# Autodesk Inventor assembly: AMR_Full_System_V1
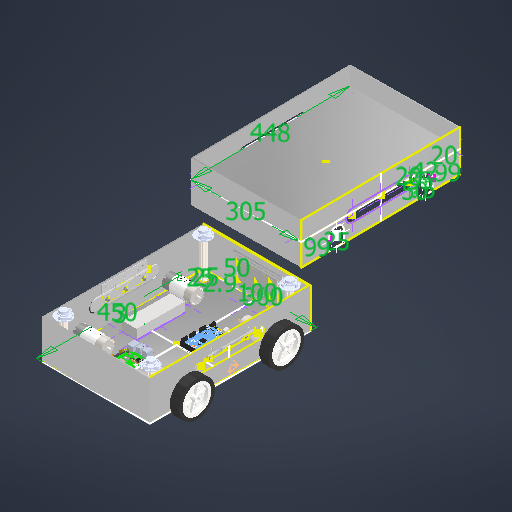
[picture p0: Inventor's stored thumbnail of the model, 512x512]
Saved by Autodesk Inventor 2026.2 (Build 302298010, 298A)
## iProperties
Created: 2026-03-25
Part Number: AMR_Full_System_V1
Document SubType Name: Assembly
Designer: Srishanth Dhondy
Author: Srishanth Dhondy
## Documents named in this file (27)
- D:\Cloud_Downloads\Srishanth\My Folder\Projects\AMR\CAD Design\hardware_cad\AMR_Full_System_V1.iam
- D:\Cloud_Downloads\Srishanth\My Folder\Projects\AMR\CAD Design\hardware_cad\AMR_Base_Box_V2.ipt
- D:\Cloud_Downloads\Srishanth\My Folder\Projects\AMR\CAD Design\hardware_cad\AMR_Top_Basket.ipt
- D:\Cloud_Downloads\Srishanth\My Folder\Projects\AMR\CAD Design\hardware_cad\Grab CAD\Wheels\Wheels v8\Wheels v8\Wheels v8.ipt
- D:\Cloud_Downloads\Srishanth\My Folder\Projects\AMR\CAD Design\hardware_cad\Grab CAD\orange-planetary-gear-dc-motor-12v-970-rpm-14-5-n-cm-pg36m555-5-2k-1.snapshot.2\Motor\Motor\Motor.ipt
- D:\Cloud_Downloads\Srishanth\My Folder\Projects\AMR\CAD Design\hardware_cad\Grab CAD\T-Slot\Aluminum Extrusion Bar\Aluminum Extrusion Bar\Aluminum Extrusion Bar.ipt
- D:\Cloud_Downloads\Srishanth\My Folder\Projects\AMR\CAD Design\hardware_cad\Grab CAD\Raspberry Pi 4\Raspberry Pi 4 Model B\Raspberry Pi 4 Model B\Raspberry Pi 4 Model B.ipt
- D:\Cloud_Downloads\Srishanth\My Folder\Projects\AMR\CAD Design\hardware_cad\AMR_Handle_Flap.ipt
- D:\Cloud_Downloads\Srishanth\My Folder\Projects\AMR\CAD Design\hardware_cad\LiPo_Battery_Dummy.ipt
- D:\Cloud_Downloads\Srishanth\My Folder\Projects\AMR\CAD Design\hardware_cad\Rear_Port_Slider.ipt
- D:\Cloud_Downloads\Srishanth\My Folder\Projects\AMR\CAD Design\hardware_cad\Grab CAD\50kg_Load_Sensor\assembly\assembly\assembly.iam
- D:\Cloud_Downloads\Srishanth\My Folder\Projects\AMR\CAD Design\hardware_cad\15205A113_Spring Hinge\15205A113_Spring Hinge\Dynamic_Hinge.iam
- C:\Users\Srishanth Dhondy\Documents\Inventor\Content Center Files\R2026\en-US\ISO 7089\ISO 7089 - 2.5 - 140 HV(1).ipt
- C:\Users\Srishanth Dhondy\Documents\Inventor\Content Center Files\R2026\en-US\ISO 4762(2)\ISO 4762 - M2.5 x 10ISO.ipt
- C:\Users\Srishanth Dhondy\Documents\Inventor\Content Center Files\R2026\en-US\ISO 7089\ISO 7089 - 3.5 - 140 HV(1).ipt
- C:\Users\Srishanth Dhondy\Documents\Inventor\Content Center Files\R2026\en-US\ISO 4762(2)\ISO 4762 - M3 x 10ISO.ipt
- C:\Users\Srishanth Dhondy\Documents\Inventor\Content Center Files\R2026\en-US\ISO 7089\ISO 7089 - 4 - 140 HV(1).ipt
- C:\Users\Srishanth Dhondy\Documents\Inventor\Content Center Files\R2026\en-US\ISO 4762(2)\ISO 4762 - M4 x 12ISO.ipt
- C:\Users\Srishanth Dhondy\Documents\Inventor\Content Center Files\R2026\en-US\DIN 985\DIN 985 - M4.ipt
- D:\Cloud_Downloads\Srishanth\My Folder\Projects\AMR\CAD Design\hardware_cad\Grab CAD\Arduino\Arduino Mega 2560 R3 v23\Arduino Mega 2560 R3 v23\Arduino Mega 2560 R3 v23.ipt
- C:\Users\Srishanth Dhondy\Documents\Inventor\Content Center Files\R2026\en-US\ISO 4762(2)\ISO 4762 - M2.5 x 16ISO.ipt
- C:\Users\Srishanth Dhondy\Documents\Inventor\Content Center Files\R2026\en-US\ISO 4032(2)\ISO 4032 - M2.5 - ISO.ipt
- D:\Cloud_Downloads\Srishanth\My Folder\Projects\AMR\CAD Design\hardware_cad\AMR_Full_System_V1\AIP\FEA\fg5kdr8u8.fins
- D:\Cloud_Downloads\Srishanth\My Folder\Projects\AMR\CAD Design\hardware_cad\AMR_Full_System_V1\AIP\FEA\fg5kdr8u8.fsat
- D:\Cloud_Downloads\Srishanth\My Folder\Projects\AMR\CAD Design\hardware_cad\AMR_Full_System_V1\AIP\FEA\fg5kdr8u8.ftes
- D:\Cloud_Downloads\Srishanth\My Folder\Projects\AMR\CAD Design\hardware_cad\AMR_Full_System_V1\AIP\FEA\fg5kdr8u8.fwiz
- D:\Cloud_Downloads\Srishanth\My Folder\Projects\AMR\CAD Design\hardware_cad\AMR_Full_System_V1\AIP\FEA\fg5kdseqo.fmsh
## Components (107 placed, 21 different names)
1. AMR_Base_Box_V2:1 — Mate:1, Rigid:11, Rigid:12, Rigid:13, Rigid:14, Slider:17, Rigid:15, Rotational:7, Rotational:8, Insert:1, Insert:2, Insert:3, Insert:4, Mate:2, Mate:4, Mate:6, Mate:8, Rotational:11, Insert:5, Insert:6, Insert:7, Insert:8, Insert:9, Insert:10, Insert:11, Insert:12, Rotational:13, Rotational:15, Insert:21, Insert:22, Insert:23, Insert:24, Insert:25, Insert:26, Insert:27, Insert:28, Rotational:19, Rotational:21, Rotational:22, Insert:63, Insert:64, Insert:65, Insert:66
2. AMR_Top_Basket:1
3. Aluminum Extrusion Bar:2 — Rigid:13, Rotational:24
4. Aluminum Extrusion Bar:3 — Rigid:12, Rigid:20
5. Aluminum Extrusion Bar:5 — Rigid:11, Rotational:25
6. Wheels v8:6
7. Raspberry Pi 4 Model B:1 — Rotational:23, Insert:71, Insert:72, Insert:73, Insert:74
8. AMR_Handle_Flap:1 — Rigid:17, Insert:43, Insert:44, Insert:45, Rigid:19
9. AMR_Handle_Flap:2 — Rotational:6, Rigid:16, Rigid:18, Insert:57, Insert:58, Insert:59
10. LiPo_Battery_Dummy:1 — Rotational:22
11. Aluminum Extrusion Bar:6 — Rigid:14, Rigid:21
12. Dynamic_Hinge:1 [sub-assembly] — Rigid:15, Rotational:6, Rigid:16, Rigid:18, Insert:51, Insert:52, Insert:53
13. Rear_Port_Slider:2 — Slider:17
14. Dynamic_Hinge:2 [sub-assembly] — Rotational:7, Rotational:8, Rigid:17, Insert:37, Insert:38, Insert:39, Rigid:19
15. ISO 7089 2.5:1 — Insert:1, Mate:3, Mate:5, Mate:7, Mate:9
16. ISO 7089 2.5:2 — Insert:2
17. ISO 7089 2.5:3 — Insert:3
18. ISO 7089 2.5:4 — Insert:4
19. ISO 4762 M2.5 x 10:1 — Mate:2, Mate:3
20. ISO 4762 M2.5 x 10:2 — Mate:4, Mate:5
21. ISO 4762 M2.5 x 10:3 — Mate:6, Mate:7
22. ISO 4762 M2.5 x 10:4 — Mate:8, Mate:9
23. Motor:5 — Rotational:11, Rotational:12
24. ISO 7089 3.5:1 — Insert:5, Insert:16
25. ISO 7089 3.5:2 — Insert:6, Insert:14
26. ISO 7089 3.5:3 — Insert:7, Insert:17
27. ISO 7089 3.5:4 — Insert:8, Insert:18
28. ISO 7089 3.5:5 — Insert:9, Insert:13
29. ISO 7089 3.5:6 — Insert:10, Insert:15
30. ISO 7089 3.5:7 — Insert:11, Insert:20
31. ISO 7089 3.5:8 — Insert:12, Insert:19
32. ISO 4762 M3 x 10:1 — Insert:13
33. ISO 4762 M3 x 10:2 — Insert:14
34. ISO 4762 M3 x 10:3 — Insert:15
35. ISO 4762 M3 x 10:4 — Insert:16
36. Wheels v8:7 — Rotational:12
37. Motor:7 — Rotational:13, Rotational:14
38. Motor:8 — Rotational:15, Rotational:16
39. ISO 4762 M3 x 10:5 — Insert:17
40. ISO 4762 M3 x 10:6 — Insert:18
41. ISO 4762 M3 x 10:7 — Insert:19
42. ISO 4762 M3 x 10:8 — Insert:20
43. Wheels v8:8 — Rotational:14
44. ISO 7089 3.5:9 — Insert:21, Insert:29
45. ISO 7089 3.5:10 — Insert:22, Insert:32
46. ISO 7089 3.5:11 — Insert:23, Insert:34
47. ISO 7089 3.5:12 — Insert:24, Insert:33
48. ISO 7089 3.5:13 — Insert:25, Insert:31
49. ISO 7089 3.5:14 — Insert:26, Insert:30
50. ISO 7089 3.5:15 — Insert:27, Insert:36
51. ISO 7089 3.5:16 — Insert:28, Insert:35
52. ISO 4762 M3 x 10:9 — Insert:29
53. ISO 4762 M3 x 10:10 — Insert:30
54. ISO 4762 M3 x 10:11 — Insert:31
55. ISO 4762 M3 x 10:12 — Insert:32
56. Wheels v8:10 — Rotational:20
57. Motor:9 — Rotational:19, Rotational:20
58. Wheels v8:11 — Rotational:16
59. ISO 4762 M3 x 10:13 — Insert:33
60. ISO 4762 M3 x 10:14 — Insert:34
61. ISO 4762 M3 x 10:15 — Insert:35
62. ISO 4762 M3 x 10:16 — Insert:36
63. ISO 7089 4:1 — Insert:37, Insert:40
64. ISO 7089 4:2 — Insert:38, Insert:42
65. ISO 7089 4:3 — Insert:39, Insert:41
66. ISO 4762 M4 x 12:1 — Insert:40
67. ISO 4762 M4 x 12:2 — Insert:41
68. ISO 4762 M4 x 12:3 — Insert:42
69. ISO 7089 4:4 — Insert:43, Insert:49
70. ISO 7089 4:5 — Insert:44, Insert:50
71. ISO 7089 4:6 — Insert:45, Insert:48
72. DIN 985 - replaced by DIN EN ISO 10511 M4:3 — Insert:48
73. DIN 985 - replaced by DIN EN ISO 10511 M4:5 — Insert:49
74. DIN 985 - replaced by DIN EN ISO 10511 M4:6 — Insert:50
75. ISO 7089 4:7 — Insert:51, Insert:54
76. ISO 7089 4:8 — Insert:52, Insert:55
77. ISO 7089 4:9 — Insert:53, Insert:56
78. ISO 4762 M4 x 12:4 — Insert:54
79. ISO 4762 M4 x 12:5 — Insert:55
80. ISO 4762 M4 x 12:6 — Insert:56
81. ISO 7089 4:10 — Insert:57, Insert:60
82. ISO 7089 4:11 — Insert:58, Insert:61
83. ISO 7089 4:12 — Insert:59, Insert:62
84. DIN 985 - replaced by DIN EN ISO 10511 M4:7 — Insert:60
85. DIN 985 - replaced by DIN EN ISO 10511 M4:8 — Insert:61
86. DIN 985 - replaced by DIN EN ISO 10511 M4:9 — Insert:62
87. Arduino Mega 2560 R3 v23:1 — Rotational:21
88. ISO 7089 2.5:5 — Insert:63, Insert:67
89. ISO 7089 2.5:6 — Insert:64, Insert:70
90. ISO 7089 2.5:7 — Insert:65, Insert:68
91. ISO 7089 2.5:8 — Insert:66, Insert:69
92. ISO 4762 M2.5 x 16:1 — Insert:67
93. ISO 4762 M2.5 x 16:2 — Insert:68, Rotational:23
94. ISO 4762 M2.5 x 16:3 — Insert:69
95. ISO 4762 M2.5 x 16:4 — Insert:70
96. ISO 7089 2.5:9 — Insert:71, Insert:75
97. ISO 7089 2.5:10 — Insert:72, Insert:76
98. ISO 7089 2.5:11 — Insert:73, Insert:77
99. ISO 7089 2.5:12 — Insert:74, Insert:78
100. ISO 4032 M2.5:1 — Insert:75
101. ISO 4032 M2.5:2 — Insert:76
102. ISO 4032 M2.5:3 — Insert:77
103. ISO 4032 M2.5:4 — Insert:78
104. assembly:5 [sub-assembly] — Rotational:24
105. assembly:6 [sub-assembly] — Rotational:25
106. assembly:7 [sub-assembly] — Rigid:21
107. assembly:8 [sub-assembly] — Rigid:20
## Relationships (114: Insert 76, RevoluteJoint 16, WeldJoint 11, Mate 9, Flush 1, TranslationJoint 1)
- Mate:1: AMR_Base_Box_V2:1
- Flush:1 (-55 mm)
- Rigid:11 [WeldJoint]: AMR_Base_Box_V2:1 ↔ Aluminum Extrusion Bar:5
- Rigid:12 [WeldJoint]: AMR_Base_Box_V2:1 ↔ Aluminum Extrusion Bar:3
- Rigid:13 [WeldJoint]: AMR_Base_Box_V2:1 ↔ Aluminum Extrusion Bar:2
- Rigid:14 [WeldJoint]: AMR_Base_Box_V2:1 ↔ Aluminum Extrusion Bar:6
- Slider:17 [TranslationJoint]: AMR_Base_Box_V2:1 ↔ Rear_Port_Slider:2
- Rigid:15 [WeldJoint]: AMR_Base_Box_V2:1 ↔ Dynamic_Hinge:1
- Rotational:6 [RevoluteJoint]: AMR_Handle_Flap:2 ↔ Dynamic_Hinge:1
- Rigid:16 [WeldJoint]: AMR_Handle_Flap:2 ↔ Dynamic_Hinge:1
- Rotational:7 [RevoluteJoint]: AMR_Base_Box_V2:1 ↔ Dynamic_Hinge:2
- Rotational:8 [RevoluteJoint]: AMR_Base_Box_V2:1 ↔ Dynamic_Hinge:2
- Rigid:17 [WeldJoint]: AMR_Handle_Flap:1 ↔ Dynamic_Hinge:2
- Insert:1: AMR_Base_Box_V2:1 ↔ ISO 7089 2.5:1
- Insert:2: AMR_Base_Box_V2:1 ↔ ISO 7089 2.5:2
- Insert:3: AMR_Base_Box_V2:1 ↔ ISO 7089 2.5:3
- Insert:4: AMR_Base_Box_V2:1 ↔ ISO 7089 2.5:4
- Mate:2: AMR_Base_Box_V2:1 ↔ ISO 4762 M2.5 x 10:1
- Mate:3: ISO 7089 2.5:1 ↔ ISO 4762 M2.5 x 10:1
- Mate:4: AMR_Base_Box_V2:1 ↔ ISO 4762 M2.5 x 10:2
- Mate:5: ISO 7089 2.5:1 ↔ ISO 4762 M2.5 x 10:2
- Mate:6: AMR_Base_Box_V2:1 ↔ ISO 4762 M2.5 x 10:3
- Mate:7: ISO 7089 2.5:1 ↔ ISO 4762 M2.5 x 10:3
- Mate:8: AMR_Base_Box_V2:1 ↔ ISO 4762 M2.5 x 10:4
- Mate:9: ISO 7089 2.5:1 ↔ ISO 4762 M2.5 x 10:4
- Rotational:11 [RevoluteJoint]: AMR_Base_Box_V2:1 ↔ Motor:5
- Insert:5: AMR_Base_Box_V2:1 ↔ ISO 7089 3.5:1
- Insert:6: AMR_Base_Box_V2:1 ↔ ISO 7089 3.5:2
- Insert:7: AMR_Base_Box_V2:1 ↔ ISO 7089 3.5:3
- Insert:8: AMR_Base_Box_V2:1 ↔ ISO 7089 3.5:4
- Insert:9: AMR_Base_Box_V2:1 ↔ ISO 7089 3.5:5
- Insert:10: AMR_Base_Box_V2:1 ↔ ISO 7089 3.5:6
- Insert:11: AMR_Base_Box_V2:1 ↔ ISO 7089 3.5:7
- Insert:12: AMR_Base_Box_V2:1 ↔ ISO 7089 3.5:8
- Insert:13: ISO 7089 3.5:5 ↔ ISO 4762 M3 x 10:1
- Insert:14: ISO 7089 3.5:2 ↔ ISO 4762 M3 x 10:2
- Insert:15: ISO 7089 3.5:6 ↔ ISO 4762 M3 x 10:3
- Insert:16: ISO 7089 3.5:1 ↔ ISO 4762 M3 x 10:4
- Rotational:12 [RevoluteJoint]: Motor:5 ↔ Wheels v8:7
- Rotational:13 [RevoluteJoint]: AMR_Base_Box_V2:1 ↔ Motor:7
- Insert:17: ISO 7089 3.5:3 ↔ ISO 4762 M3 x 10:5
- Insert:18: ISO 7089 3.5:4 ↔ ISO 4762 M3 x 10:6
- Insert:19: ISO 7089 3.5:8 ↔ ISO 4762 M3 x 10:7
- Insert:20: ISO 7089 3.5:7 ↔ ISO 4762 M3 x 10:8
- Rotational:14 [RevoluteJoint]: Motor:7 ↔ Wheels v8:8
- Rotational:15 [RevoluteJoint]: AMR_Base_Box_V2:1 ↔ Motor:8
- Insert:21: AMR_Base_Box_V2:1 ↔ ISO 7089 3.5:9
- Insert:22: AMR_Base_Box_V2:1 ↔ ISO 7089 3.5:10
- Insert:23: AMR_Base_Box_V2:1 ↔ ISO 7089 3.5:11
- Insert:24: AMR_Base_Box_V2:1 ↔ ISO 7089 3.5:12
- Insert:25: AMR_Base_Box_V2:1 ↔ ISO 7089 3.5:13
- Insert:26: AMR_Base_Box_V2:1 ↔ ISO 7089 3.5:14
- Insert:27: AMR_Base_Box_V2:1 ↔ ISO 7089 3.5:15
- Insert:28: AMR_Base_Box_V2:1 ↔ ISO 7089 3.5:16
- Insert:29: ISO 7089 3.5:9 ↔ ISO 4762 M3 x 10:9
- Insert:30: ISO 7089 3.5:14 ↔ ISO 4762 M3 x 10:10
- Insert:31: ISO 7089 3.5:13 ↔ ISO 4762 M3 x 10:11
- Insert:32: ISO 7089 3.5:10 ↔ ISO 4762 M3 x 10:12
- Rotational:16 [RevoluteJoint]: Motor:8 ↔ Wheels v8:11
- Rotational:19 [RevoluteJoint]: AMR_Base_Box_V2:1 ↔ Motor:9
- Insert:33: ISO 7089 3.5:12 ↔ ISO 4762 M3 x 10:13
- Insert:34: ISO 7089 3.5:11 ↔ ISO 4762 M3 x 10:14
- Insert:35: ISO 7089 3.5:16 ↔ ISO 4762 M3 x 10:15
- Insert:36: ISO 7089 3.5:15 ↔ ISO 4762 M3 x 10:16
- Rotational:20 [RevoluteJoint]: Wheels v8:10 ↔ Motor:9
- Insert:37: Dynamic_Hinge:2 ↔ ISO 7089 4:1
- Insert:38: Dynamic_Hinge:2 ↔ ISO 7089 4:2
- Insert:39: Dynamic_Hinge:2 ↔ ISO 7089 4:3
- Insert:40: ISO 7089 4:1 ↔ ISO 4762 M4 x 12:1
- Insert:41: ISO 7089 4:3 ↔ ISO 4762 M4 x 12:2
- Insert:42: ISO 7089 4:2 ↔ ISO 4762 M4 x 12:3
- Insert:43: AMR_Handle_Flap:1 ↔ ISO 7089 4:4
- Insert:44: AMR_Handle_Flap:1 ↔ ISO 7089 4:5
- Insert:45: AMR_Handle_Flap:1 ↔ ISO 7089 4:6
- Insert:48: ISO 7089 4:6 ↔ DIN 985 - replaced by DIN EN ISO 10511 M4:3
- Insert:49: ISO 7089 4:4 ↔ DIN 985 - replaced by DIN EN ISO 10511 M4:5
- Insert:50: ISO 7089 4:5 ↔ DIN 985 - replaced by DIN EN ISO 10511 M4:6
- Rigid:18 [WeldJoint]: AMR_Handle_Flap:2 ↔ Dynamic_Hinge:1
- Rigid:19 [WeldJoint]: AMR_Handle_Flap:1 ↔ Dynamic_Hinge:2
- Insert:51: Dynamic_Hinge:1 ↔ ISO 7089 4:7
- Insert:52: Dynamic_Hinge:1 ↔ ISO 7089 4:8
- Insert:53: Dynamic_Hinge:1 ↔ ISO 7089 4:9
- Insert:54: ISO 7089 4:7 ↔ ISO 4762 M4 x 12:4
- Insert:55: ISO 7089 4:8 ↔ ISO 4762 M4 x 12:5
- Insert:56: ISO 7089 4:9 ↔ ISO 4762 M4 x 12:6
- Insert:57: AMR_Handle_Flap:2 ↔ ISO 7089 4:10
- Insert:58: AMR_Handle_Flap:2 ↔ ISO 7089 4:11
- Insert:59: AMR_Handle_Flap:2 ↔ ISO 7089 4:12
- Insert:60: ISO 7089 4:10 ↔ DIN 985 - replaced by DIN EN ISO 10511 M4:7
- Insert:61: ISO 7089 4:11 ↔ DIN 985 - replaced by DIN EN ISO 10511 M4:8
- Insert:62: ISO 7089 4:12 ↔ DIN 985 - replaced by DIN EN ISO 10511 M4:9
- Rotational:21 [RevoluteJoint]: AMR_Base_Box_V2:1 ↔ Arduino Mega 2560 R3 v23:1
- Rotational:22 [RevoluteJoint]: AMR_Base_Box_V2:1 ↔ LiPo_Battery_Dummy:1
- Insert:63: AMR_Base_Box_V2:1 ↔ ISO 7089 2.5:5
- Insert:64: AMR_Base_Box_V2:1 ↔ ISO 7089 2.5:6
- Insert:65: AMR_Base_Box_V2:1 ↔ ISO 7089 2.5:7
- Insert:66: AMR_Base_Box_V2:1 ↔ ISO 7089 2.5:8
- Insert:67: ISO 7089 2.5:5 ↔ ISO 4762 M2.5 x 16:1
- Insert:68: ISO 7089 2.5:7 ↔ ISO 4762 M2.5 x 16:2
- Insert:69: ISO 7089 2.5:8 ↔ ISO 4762 M2.5 x 16:3
- Insert:70: ISO 7089 2.5:6 ↔ ISO 4762 M2.5 x 16:4
- Rotational:23 [RevoluteJoint]: Raspberry Pi 4 Model B:1 ↔ ISO 4762 M2.5 x 16:2
- Insert:71: Raspberry Pi 4 Model B:1 ↔ ISO 7089 2.5:9
- Insert:72: Raspberry Pi 4 Model B:1 ↔ ISO 7089 2.5:10
- Insert:73: Raspberry Pi 4 Model B:1 ↔ ISO 7089 2.5:11
- Insert:74: Raspberry Pi 4 Model B:1 ↔ ISO 7089 2.5:12
- Insert:75: ISO 7089 2.5:9 ↔ ISO 4032 M2.5:1
- Insert:76: ISO 7089 2.5:10 ↔ ISO 4032 M2.5:2
- Insert:77: ISO 7089 2.5:11 ↔ ISO 4032 M2.5:3
- Insert:78: ISO 7089 2.5:12 ↔ ISO 4032 M2.5:4
- Rotational:24 [RevoluteJoint]: Aluminum Extrusion Bar:2 ↔ assembly:5
- Rotational:25 [RevoluteJoint]: Aluminum Extrusion Bar:5 ↔ assembly:6
- Rigid:20 [WeldJoint]: Aluminum Extrusion Bar:3 ↔ assembly:8
- Rigid:21 [WeldJoint]: Aluminum Extrusion Bar:6 ↔ assembly:7
## Named parameters: sa_0 = 8896.44, sa_1 = 8896.44, sa_2 = 8896.44
note: some values were not read from the file. Shown as the stored number, unit unknown: "sa_0", "sa_1", "sa_2".
